# Autodesk Inventor assembly: Assembly
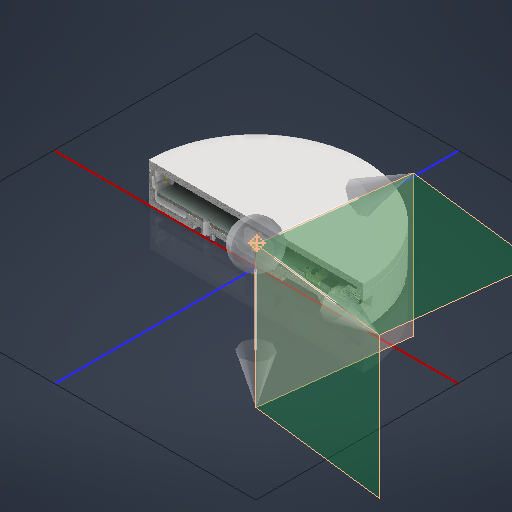
[picture p0: Inventor's stored thumbnail of the model, 512x512]
Saved by Autodesk Inventor 2026 (Build 300175050, 175E)
## iProperties
Created: 2025-07-28
Part Number: Assembly
Document SubType Name: Assembly
Designer: bruno
Author: bruno
## Documents named in this file (4)
- C:\Users\bruno\prod-alarma-cebado\enclosure\Assembly.iam
- C:\Users\bruno\prod-alarma-cebado\enclosure\housing.ipt
- C:\Users\bruno\prod-alarma-cebado\enclosure\board\board\pcb_board.iam
- C:\Users\bruno\prod-alarma-cebado\enclosure\plate.ipt
## Components (3 placed, 3 different names)
1. housing:1 — Flush:1, Flush:2, Flush:3, Mate:4
2. pcb_board:1 [sub-assembly] — Mate:1, Flush:4
3. plate:1 — Flush:5, Mate:2, Mate:3, Mate:4
## Relationships (9: Flush 5, Mate 4)
- Flush:1: housing:1
- Flush:2: housing:1
- Flush:3: housing:1
- Mate:1: pcb_board:1
- Flush:4: pcb_board:1
- Flush:5: plate:1
- Mate:2: plate:1
- Mate:3: plate:1
- Mate:4: housing:1 ↔ plate:1
